# Autodesk Inventor assembly: use this - gimme that tech award
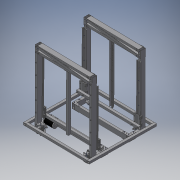
[picture p0: Inventor's stored thumbnail of the model, 180x180]
Saved by Autodesk Inventor 2018 (Build 220112000, 112)
## iProperties
Created: 2019-01-10
Part Number: use this - gimme that tech award
Document SubType Name: Assembly
Designer: maste
Author: maste
## Documents named in this file (9)
- C:\Users\maste\OneDrive\Documents\GitHub\2019CAD\Drivebase but Calvin is a mad man\use this - gimme that tech award.iam
- C:\Users\maste\OneDrive\Documents\GitHub\2019CAD\Drivebase but Calvin is a mad man\Slidey Mecanum L thing V2.iam
- C:\Users\maste\OneDrive\Documents\GitHub\2019CAD\Drivebase but Calvin is a mad man\WW_10_40_10_AL_2.ipt
- C:\Users\maste\OneDrive\Documents\GitHub\2019CAD\Drivebase but Calvin is a mad man\1x1 29in.ipt
- C:\Users\maste\OneDrive\Documents\GitHub\2019CAD\Drivebase but Calvin is a mad man\1x1 27in.ipt
- C:\Users\maste\OneDrive\Documents\GitHub\2019CAD\Drivebase but Calvin is a mad man\CIM_Motor_217-2000.ipt
- C:\Users\maste\OneDrive\Documents\GitHub\2019CAD\Drivebase but Calvin is a mad man\91292A197_TYPE 18-8 SS SOCKET HEAD CAP SCREW (1).ipt
- C:\Users\maste\OneDrive\Documents\GitHub\2019CAD\Drivebase but Calvin is a mad man\1x1 27 362in.ipt
- C:\Users\maste\OneDrive\Documents\GitHub\2019CAD\Drivebase but Calvin is a mad man\93625A200_TYPE 18-8 STAINLESS STL NYLON-INSERT LOCKNUT.ipt
## Components (29 placed, 8 different names)
1. Slidey Mecanum L thing V2:1 [sub-assembly] — Mate:59, Mate:60, Mate:61, Mate:62, Flush:1, Mate:74, Mate:75, Flush:5, Flush:6
2. Slidey Mecanum L thing V2:2 [sub-assembly] — Mate:55, Mate:56, Mate:57, Mate:58, Flush:2, Mate:72, Mate:73, Flush:3, Flush:4
3. WW_10_40_10_AL_2:1 — Mate:57, Mate:58, Flush:3, Mate:76, Mate:77, Mate:78, Mate:79
4. WW_10_40_10_AL_2:2 — Mate:59, Mate:60, Flush:5, Mate:88, Mate:89, Mate:90, Mate:91, Mate:92, Angle:1
5. WW_10_40_10_AL_2:3 — Mate:61, Mate:62, Flush:6, Mate:84, Mate:85, Mate:86, Mate:87
6. WW_10_40_10_AL_2:4 — Mate:55, Mate:56, Flush:4, Mate:80, Mate:81, Mate:82, Mate:83, Mate:94, Angle:2
7. 1x1 29in:1 — Mate:69, Mate:70, Mate:71, Mate:74, Mate:75
8. 1x1 29in:2 — Mate:63, Mate:64, Mate:65, Mate:66, Mate:67, Mate:68, Mate:72, Mate:73
9. 1x1 27in:1 — Mate:66, Mate:67, Mate:68, Mate:69, Mate:70, Mate:71, Flush:2
10. 1x1 27in:2 — Mate:63, Mate:64, Mate:65, Flush:1
11. CIM_Motor_217-2000:1
12. 91292A197_TYPE 18-8 SS SOCKET HEAD CAP SCREW (1):1 — Mate:76, Mate:77, Mate:106
13. 91292A197_TYPE 18-8 SS SOCKET HEAD CAP SCREW (1):2 — Mate:78, Mate:79, Mate:107
14. 91292A197_TYPE 18-8 SS SOCKET HEAD CAP SCREW (1):3 — Mate:80, Mate:81, Mate:110
15. 91292A197_TYPE 18-8 SS SOCKET HEAD CAP SCREW (1):4 — Mate:82, Mate:83, Mate:95, Mate:111
16. 91292A197_TYPE 18-8 SS SOCKET HEAD CAP SCREW (1):5 — Mate:84, Mate:85, Mate:103
17. 91292A197_TYPE 18-8 SS SOCKET HEAD CAP SCREW (1):6 — Mate:86, Mate:87, Mate:102
18. 91292A197_TYPE 18-8 SS SOCKET HEAD CAP SCREW (1):7 — Mate:90, Mate:91, Mate:99
19. 91292A197_TYPE 18-8 SS SOCKET HEAD CAP SCREW (1):8 — Mate:88, Mate:89, Mate:93, Mate:98
20. 1x1 27 362in:1 — Mate:92, Mate:93, Angle:1, Mate:96, Mate:97, Mate:100, Mate:101
21. 1x1 27 362in:2 — Mate:94, Mate:95, Angle:2, Mate:104, Mate:105, Mate:108, Mate:109
22. 93625A200_TYPE 18-8 STAINLESS STL NYLON-INSERT LOCKNUT:1 — Mate:108, Mate:111
23. 93625A200_TYPE 18-8 STAINLESS STL NYLON-INSERT LOCKNUT:2 — Mate:109, Mate:110
24. 93625A200_TYPE 18-8 STAINLESS STL NYLON-INSERT LOCKNUT:3 — Mate:104, Mate:106
25. 93625A200_TYPE 18-8 STAINLESS STL NYLON-INSERT LOCKNUT:4 — Mate:105, Mate:107
26. 93625A200_TYPE 18-8 STAINLESS STL NYLON-INSERT LOCKNUT:6 — Mate:97, Mate:99
27. 93625A200_TYPE 18-8 STAINLESS STL NYLON-INSERT LOCKNUT:7 — Mate:96, Mate:98
28. 93625A200_TYPE 18-8 STAINLESS STL NYLON-INSERT LOCKNUT:8 — Mate:101, Mate:103
29. 93625A200_TYPE 18-8 STAINLESS STL NYLON-INSERT LOCKNUT:9 — Mate:100, Mate:102
## Relationships (65: Mate 57, Flush 6, Angle 2)
- Mate:55: Slidey Mecanum L thing V2:2 ↔ WW_10_40_10_AL_2:4
- Mate:56: Slidey Mecanum L thing V2:2 ↔ WW_10_40_10_AL_2:4
- Mate:57: Slidey Mecanum L thing V2:2 ↔ WW_10_40_10_AL_2:1
- Mate:58: Slidey Mecanum L thing V2:2 ↔ WW_10_40_10_AL_2:1
- Mate:59: Slidey Mecanum L thing V2:1 ↔ WW_10_40_10_AL_2:2
- Mate:60: Slidey Mecanum L thing V2:1 ↔ WW_10_40_10_AL_2:2
- Mate:61: Slidey Mecanum L thing V2:1 ↔ WW_10_40_10_AL_2:3
- Mate:62: Slidey Mecanum L thing V2:1 ↔ WW_10_40_10_AL_2:3
- Mate:63: 1x1 29in:2 ↔ 1x1 27in:2
- Mate:64: 1x1 29in:2 ↔ 1x1 27in:2
- Mate:65: 1x1 29in:2 ↔ 1x1 27in:2
- Mate:66: 1x1 29in:2 ↔ 1x1 27in:1
- Mate:67: 1x1 29in:2 ↔ 1x1 27in:1
- Mate:68: 1x1 29in:2 ↔ 1x1 27in:1
- Mate:69: 1x1 29in:1 ↔ 1x1 27in:1
- Mate:70: 1x1 29in:1 ↔ 1x1 27in:1
- Mate:71: 1x1 29in:1 ↔ 1x1 27in:1
- Flush:1 (101.6 mm): Slidey Mecanum L thing V2:1 ↔ 1x1 27in:2
- Flush:2 (-101.6 mm): Slidey Mecanum L thing V2:2 ↔ 1x1 27in:1
- Mate:72 (25.4 mm): Slidey Mecanum L thing V2:2 ↔ 1x1 29in:2
- Mate:73: Slidey Mecanum L thing V2:2 ↔ 1x1 29in:2
- Mate:74: Slidey Mecanum L thing V2:1 ↔ 1x1 29in:1
- Mate:75 (25.4 mm): Slidey Mecanum L thing V2:1 ↔ 1x1 29in:1
- Flush:3: Slidey Mecanum L thing V2:2 ↔ WW_10_40_10_AL_2:1
- Flush:4: Slidey Mecanum L thing V2:2 ↔ WW_10_40_10_AL_2:4
- Flush:5: Slidey Mecanum L thing V2:1 ↔ WW_10_40_10_AL_2:2
- Flush:6: Slidey Mecanum L thing V2:1 ↔ WW_10_40_10_AL_2:3
- Mate:76: WW_10_40_10_AL_2:1 ↔ 91292A197_TYPE 18-8 SS SOCKET HEAD CAP SCREW (1):1
- Mate:77: WW_10_40_10_AL_2:1 ↔ 91292A197_TYPE 18-8 SS SOCKET HEAD CAP SCREW (1):1
- Mate:78: WW_10_40_10_AL_2:1 ↔ 91292A197_TYPE 18-8 SS SOCKET HEAD CAP SCREW (1):2
- Mate:79: WW_10_40_10_AL_2:1 ↔ 91292A197_TYPE 18-8 SS SOCKET HEAD CAP SCREW (1):2
- Mate:80: WW_10_40_10_AL_2:4 ↔ 91292A197_TYPE 18-8 SS SOCKET HEAD CAP SCREW (1):3
- Mate:81: WW_10_40_10_AL_2:4 ↔ 91292A197_TYPE 18-8 SS SOCKET HEAD CAP SCREW (1):3
- Mate:82: WW_10_40_10_AL_2:4 ↔ 91292A197_TYPE 18-8 SS SOCKET HEAD CAP SCREW (1):4
- Mate:83: WW_10_40_10_AL_2:4 ↔ 91292A197_TYPE 18-8 SS SOCKET HEAD CAP SCREW (1):4
- Mate:84: WW_10_40_10_AL_2:3 ↔ 91292A197_TYPE 18-8 SS SOCKET HEAD CAP SCREW (1):5
- Mate:85: WW_10_40_10_AL_2:3 ↔ 91292A197_TYPE 18-8 SS SOCKET HEAD CAP SCREW (1):5
- Mate:86: WW_10_40_10_AL_2:3 ↔ 91292A197_TYPE 18-8 SS SOCKET HEAD CAP SCREW (1):6
- Mate:87: WW_10_40_10_AL_2:3 ↔ 91292A197_TYPE 18-8 SS SOCKET HEAD CAP SCREW (1):6
- Mate:88: WW_10_40_10_AL_2:2 ↔ 91292A197_TYPE 18-8 SS SOCKET HEAD CAP SCREW (1):8
- Mate:89: WW_10_40_10_AL_2:2 ↔ 91292A197_TYPE 18-8 SS SOCKET HEAD CAP SCREW (1):8
- Mate:90: WW_10_40_10_AL_2:2 ↔ 91292A197_TYPE 18-8 SS SOCKET HEAD CAP SCREW (1):7
- Mate:91: WW_10_40_10_AL_2:2 ↔ 91292A197_TYPE 18-8 SS SOCKET HEAD CAP SCREW (1):7
- Mate:92: WW_10_40_10_AL_2:2 ↔ 1x1 27 362in:1
- Mate:93: 91292A197_TYPE 18-8 SS SOCKET HEAD CAP SCREW (1):8 ↔ 1x1 27 362in:1
- Angle:1 (-90 deg): WW_10_40_10_AL_2:2 ↔ 1x1 27 362in:1
- Mate:94: WW_10_40_10_AL_2:4 ↔ 1x1 27 362in:2
- Mate:95: 91292A197_TYPE 18-8 SS SOCKET HEAD CAP SCREW (1):4 ↔ 1x1 27 362in:2
- Angle:2 (-90 deg): WW_10_40_10_AL_2:4 ↔ 1x1 27 362in:2
- Mate:96: 1x1 27 362in:1 ↔ 93625A200_TYPE 18-8 STAINLESS STL NYLON-INSERT LOCKNUT:7
- Mate:97: 1x1 27 362in:1 ↔ 93625A200_TYPE 18-8 STAINLESS STL NYLON-INSERT LOCKNUT:6
- Mate:98: 91292A197_TYPE 18-8 SS SOCKET HEAD CAP SCREW (1):8 ↔ 93625A200_TYPE 18-8 STAINLESS STL NYLON-INSERT LOCKNUT:7
- Mate:99: 91292A197_TYPE 18-8 SS SOCKET HEAD CAP SCREW (1):7 ↔ 93625A200_TYPE 18-8 STAINLESS STL NYLON-INSERT LOCKNUT:6
- Mate:100: 1x1 27 362in:1 ↔ 93625A200_TYPE 18-8 STAINLESS STL NYLON-INSERT LOCKNUT:9
- Mate:101: 1x1 27 362in:1 ↔ 93625A200_TYPE 18-8 STAINLESS STL NYLON-INSERT LOCKNUT:8
- Mate:102: 91292A197_TYPE 18-8 SS SOCKET HEAD CAP SCREW (1):6 ↔ 93625A200_TYPE 18-8 STAINLESS STL NYLON-INSERT LOCKNUT:9
- Mate:103: 91292A197_TYPE 18-8 SS SOCKET HEAD CAP SCREW (1):5 ↔ 93625A200_TYPE 18-8 STAINLESS STL NYLON-INSERT LOCKNUT:8
- Mate:104: 1x1 27 362in:2 ↔ 93625A200_TYPE 18-8 STAINLESS STL NYLON-INSERT LOCKNUT:3
- Mate:105: 1x1 27 362in:2 ↔ 93625A200_TYPE 18-8 STAINLESS STL NYLON-INSERT LOCKNUT:4
- Mate:106: 91292A197_TYPE 18-8 SS SOCKET HEAD CAP SCREW (1):1 ↔ 93625A200_TYPE 18-8 STAINLESS STL NYLON-INSERT LOCKNUT:3
- Mate:107: 91292A197_TYPE 18-8 SS SOCKET HEAD CAP SCREW (1):2 ↔ 93625A200_TYPE 18-8 STAINLESS STL NYLON-INSERT LOCKNUT:4
- Mate:108: 1x1 27 362in:2 ↔ 93625A200_TYPE 18-8 STAINLESS STL NYLON-INSERT LOCKNUT:1
- Mate:109: 1x1 27 362in:2 ↔ 93625A200_TYPE 18-8 STAINLESS STL NYLON-INSERT LOCKNUT:2
- Mate:110: 91292A197_TYPE 18-8 SS SOCKET HEAD CAP SCREW (1):3 ↔ 93625A200_TYPE 18-8 STAINLESS STL NYLON-INSERT LOCKNUT:2
- Mate:111: 91292A197_TYPE 18-8 SS SOCKET HEAD CAP SCREW (1):4 ↔ 93625A200_TYPE 18-8 STAINLESS STL NYLON-INSERT LOCKNUT:1
